# Autodesk Inventor assembly: endAssembly
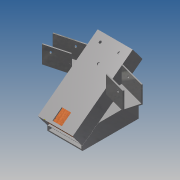
[picture p0: Inventor's stored thumbnail of the model, 180x180]
Saved by Autodesk Inventor 2014 SP1 (Build 180222100, 222)
## iProperties
Created: 2013-12-03
Part Number: endAssembly
Document SubType Name: Assembly
Designer: Dave
Author: Dave
## Documents named in this file (7)
- C:\Users\Dave\Desktop\hera-cad\support\endAssembly.iam
- C:\Users\Dave\Desktop\hera-cad\support\endHoriz.ipt
- C:\Users\Dave\Desktop\hera-cad\support\end37.ipt
- C:\Users\Dave\Desktop\hera-cad\support\endWoodblock.ipt
- C:\Users\Dave\Desktop\hera-cad\support\endChannel.ipt
- C:\Users\Dave\Desktop\hera-cad\support\endBlock.ipt
- C:\Users\Dave\Desktop\hera-cad\support\endChannel_MIR.ipt
## Components (6 placed, 6 different names)
1. endHoriz:1 — Mate:1, Flush:3, Mate:11, Flush:4, Flush:5, Mate:12
2. end37:1 — Mate:1, Flush:3, Mate:8, Mate:9, Mate:10, Flush:6
3. endWoodblock:1 — Mate:8, Mate:9, Mate:10
4. endChannel:1 — Mate:11, Flush:4, Flush:5
5. endBlock:1 — Mate:12
6. endChannel_MIR:1
## Relationships (10: Mate 6, Flush 4)
- Mate:1: endHoriz:1 ↔ end37:1
- Flush:3: endHoriz:1 ↔ end37:1
- Mate:8: end37:1 ↔ endWoodblock:1
- Mate:9: end37:1 ↔ endWoodblock:1
- Mate:10: end37:1 ↔ endWoodblock:1
- Mate:11: endHoriz:1 ↔ endChannel:1
- Flush:4 (-63.5 mm): endHoriz:1 ↔ endChannel:1
- Flush:5 (-60.198 mm): endHoriz:1 ↔ endChannel:1
- Mate:12: endHoriz:1 ↔ endBlock:1
- Flush:6 (-47.498 mm): end37:1
